# Autodesk Inventor assembly: Cadenas de soporte de bandejas 1.1
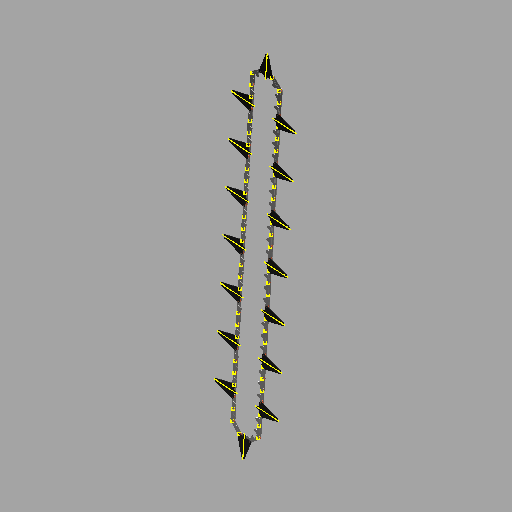
[picture p0: Inventor's stored thumbnail of the model, 512x512]
Saved by Autodesk Inventor 2024.3 (Build 283343010, 343A)
## iProperties
Created: 2025-05-22
Part Number: Cadenas de soporte de bandejas 1.1
Document SubType Name: Weldment
Designer: Gary
Weld Material: Welded Aluminum-6061
Author: Gary
## Documents named in this file (7)
- D:\OneDrive - Universidad Tecnologica del Peru\Desktop\Proyecto Final (Avance) Elementos de maquinas\Estructura principal\Cadenas de soporte de bandejas 1.1.iam
- D:\OneDrive - Universidad Tecnologica del Peru\Desktop\Proyecto Final (Avance) Elementos de maquinas\Estructura principal\Eslabon de arrastre posterior.ipt
- D:\OneDrive - Universidad Tecnologica del Peru\Desktop\Proyecto Final (Avance) Elementos de maquinas\Estructura principal\Eslabon de arrastre externo.ipt
- D:\OneDrive - Universidad Tecnologica del Peru\Desktop\Proyecto Final (Avance) Elementos de maquinas\Estructura principal\Eslabon de arrastre interno.ipt
- D:\OneDrive - Universidad Tecnologica del Peru\Desktop\Proyecto Final (Avance) Elementos de maquinas\Estructura principal\Rodillo Guia de Cadena.ipt
- D:\OneDrive - Universidad Tecnologica del Peru\Desktop\Proyecto Final (Avance) Elementos de maquinas\Estructura principal\Pasador Eslabones de Cadena.ipt
- D:\OneDrive - Universidad Tecnologica del Peru\Desktop\Proyecto Final (Avance) Elementos de maquinas\Estructura principal\Eslabon de arranque y movimiento bandeja.ipt
## Components (256 placed, 6 different names)
1. Eslabon de arrastre posterior:1 — Insert:12, Insert:13, Insert:16, Insert:283
2. Eslabon de arrastre externo:1 — Insert:4, Mate:1, Insert:6, Insert:7
3. Eslabon de arrastre interno:1 — Insert:3, Insert:4, Insert:5, Insert:353
4. Rodillo Guia de Cadena:1 — Insert:3, Insert:12
5. Pasador Eslabones de Cadena:1 — Insert:354
6. Pasador Eslabones de Cadena:2 — Insert:7
7. Pasador Eslabones de Cadena:3 — Mate:1
8. Pasador Eslabones de Cadena:4 — Insert:356
9. Rodillo Guia de Cadena:2 — Insert:5, Insert:13
10. Rodillo Guia de Cadena:3 — Insert:8, Insert:14
11. Rodillo Guia de Cadena:4 — Insert:11, Insert:15
12. Eslabon de arrastre interno:2 — Insert:6, Insert:8, Insert:11, Insert:355
13. Eslabon de arrastre posterior:2 — Insert:14, Insert:15, Insert:17, Insert:282
14. Eslabon de arrastre posterior:5 — Insert:16, Insert:17
15. Eslabon de arrastre posterior:9 — Insert:281
16. Eslabon de arrastre externo:2
17. Eslabon de arrastre interno:5 — Insert:357
18. Rodillo Guia de Cadena:9
19. Pasador Eslabones de Cadena:5 — Insert:358
20. Pasador Eslabones de Cadena:6
21. Pasador Eslabones de Cadena:7
22. Pasador Eslabones de Cadena:8 — Insert:360
23. Rodillo Guia de Cadena:10
24. Rodillo Guia de Cadena:11
25. Rodillo Guia de Cadena:12
26. Eslabon de arrastre interno:6 — Insert:359
27. Eslabon de arrastre posterior:10 — Insert:280
28. Eslabon de arrastre posterior:11
29. Eslabon de arrastre posterior:12 — Insert:279
30. Eslabon de arrastre externo:3
31. Eslabon de arrastre interno:7 — Insert:361
32. Rodillo Guia de Cadena:13
33. Pasador Eslabones de Cadena:9 — Insert:362
34. Pasador Eslabones de Cadena:10
35. Pasador Eslabones de Cadena:11
36. Pasador Eslabones de Cadena:12 — Insert:364
37. Rodillo Guia de Cadena:14
38. Rodillo Guia de Cadena:15
39. Rodillo Guia de Cadena:16
40. Eslabon de arrastre interno:8 — Insert:363
41. Eslabon de arrastre posterior:13 — Insert:278
42. Eslabon de arrastre posterior:14
43. Eslabon de arrastre posterior:15 — Insert:277
44. Eslabon de arrastre externo:4
45. Eslabon de arrastre interno:9 — Insert:365
46. Rodillo Guia de Cadena:17
47. Pasador Eslabones de Cadena:13
48. Pasador Eslabones de Cadena:14
49. Pasador Eslabones de Cadena:15 — Insert:303
50. Rodillo Guia de Cadena:18
51. Rodillo Guia de Cadena:19
52. Rodillo Guia de Cadena:20
53. Eslabon de arrastre interno:10 — Insert:306
54. Eslabon de arrastre posterior:16 — Insert:275
55. Eslabon de arrastre posterior:17
56. Eslabon de arrastre posterior:18 — Insert:276
57. Eslabon de arrastre externo:5
58. Eslabon de arrastre interno:11 — Insert:305
59. Rodillo Guia de Cadena:21
60. Pasador Eslabones de Cadena:16
61. Pasador Eslabones de Cadena:17
62. Pasador Eslabones de Cadena:18 — Insert:308
63. Rodillo Guia de Cadena:22
64. Rodillo Guia de Cadena:23
65. Rodillo Guia de Cadena:24
66. Eslabon de arrastre interno:12 — Insert:310
67. Eslabon de arrastre posterior:19 — Insert:273
68. Eslabon de arrastre posterior:20
69. Pasador Eslabones de Cadena:19 — Insert:366
70. Pasador Eslabones de Cadena:20 — Insert:304
71. Pasador Eslabones de Cadena:21 — Insert:352
72. Eslabon de arrastre posterior:21 — Insert:290
73. Eslabon de arrastre externo:6
74. Eslabon de arrastre interno:13 — Insert:332
75. Rodillo Guia de Cadena:25
76. Pasador Eslabones de Cadena:22 — Insert:334
77. Pasador Eslabones de Cadena:23
78. Pasador Eslabones de Cadena:24
79. Pasador Eslabones de Cadena:25 — Insert:336
80. Rodillo Guia de Cadena:26
81. Rodillo Guia de Cadena:27
82. Rodillo Guia de Cadena:28
83. Eslabon de arrastre interno:14 — Insert:335
84. Eslabon de arrastre posterior:22 — Mate:18
85. Eslabon de arrastre posterior:23
86. Eslabon de arrastre posterior:24 — Mate:17
87. Eslabon de arrastre externo:7
88. Eslabon de arrastre interno:15 — Insert:337
89. Rodillo Guia de Cadena:29
90. Pasador Eslabones de Cadena:26 — Insert:338
91. Pasador Eslabones de Cadena:27
92. Pasador Eslabones de Cadena:28
93. Pasador Eslabones de Cadena:29 — Insert:340
94. Rodillo Guia de Cadena:30
95. Rodillo Guia de Cadena:31
96. Rodillo Guia de Cadena:32
97. Eslabon de arrastre interno:16 — Insert:339
98. Eslabon de arrastre posterior:25 — Insert:288
99. Eslabon de arrastre posterior:26
100. Eslabon de arrastre posterior:27 — Insert:289
101. Eslabon de arrastre externo:8
102. Eslabon de arrastre interno:17 — Insert:341
103. Rodillo Guia de Cadena:33
104. Pasador Eslabones de Cadena:30 — Insert:342
105. Pasador Eslabones de Cadena:31
106. Pasador Eslabones de Cadena:32
107. Pasador Eslabones de Cadena:33 — Insert:344
108. Rodillo Guia de Cadena:34
109. Rodillo Guia de Cadena:35
110. Rodillo Guia de Cadena:36
111. Eslabon de arrastre interno:18 — Insert:343
112. Eslabon de arrastre posterior:28 — Insert:286
113. Eslabon de arrastre posterior:29
114. Eslabon de arrastre posterior:30 — Insert:287
115. Eslabon de arrastre externo:9
116. Eslabon de arrastre interno:19 — Insert:345
117. Rodillo Guia de Cadena:37
118. Pasador Eslabones de Cadena:34
119. Pasador Eslabones de Cadena:35
120. Pasador Eslabones de Cadena:36 — Insert:348
121. Rodillo Guia de Cadena:38
122. Rodillo Guia de Cadena:39
123. Rodillo Guia de Cadena:40
124. Eslabon de arrastre interno:20 — Insert:347
125. Eslabon de arrastre posterior:31 — Insert:284
126. Eslabon de arrastre posterior:32
127. Eslabon de arrastre posterior:33 — Insert:285
128. Eslabon de arrastre externo:10
129. Eslabon de arrastre interno:21 — Insert:349
130. Rodillo Guia de Cadena:41
131. Pasador Eslabones de Cadena:37
132. Pasador Eslabones de Cadena:38
133. Rodillo Guia de Cadena:42
134. Rodillo Guia de Cadena:43
135. Rodillo Guia de Cadena:44
136. Eslabon de arrastre interno:22 — Insert:351
137. Eslabon de arrastre posterior:34 — Insert:300
138. Eslabon de arrastre posterior:35
139. Pasador Eslabones de Cadena:39 — Insert:346
140. Pasador Eslabones de Cadena:40 — Insert:350
141. Eslabon de arrastre posterior:36 — Insert:302
142. Eslabon de arrastre externo:11
143. Eslabon de arrastre interno:23 — Insert:313
144. Rodillo Guia de Cadena:45
145. Pasador Eslabones de Cadena:41 — Insert:312
146. Pasador Eslabones de Cadena:42
147. Pasador Eslabones de Cadena:43
148. Pasador Eslabones de Cadena:44 — Insert:317
149. Rodillo Guia de Cadena:46
150. Rodillo Guia de Cadena:47
151. Rodillo Guia de Cadena:48
152. Eslabon de arrastre interno:24 — Insert:315
153. Eslabon de arrastre posterior:37 — Insert:299
154. Eslabon de arrastre posterior:38
155. Eslabon de arrastre posterior:39 — Insert:298
156. Eslabon de arrastre externo:12
157. Eslabon de arrastre interno:25 — Insert:316
158. Rodillo Guia de Cadena:49
159. Pasador Eslabones de Cadena:45 — Insert:318
160. Pasador Eslabones de Cadena:46
161. Pasador Eslabones de Cadena:47
162. Pasador Eslabones de Cadena:48 — Insert:321
163. Rodillo Guia de Cadena:50
164. Rodillo Guia de Cadena:51
165. Rodillo Guia de Cadena:52
166. Eslabon de arrastre interno:26 — Insert:319
167. Eslabon de arrastre posterior:40 — Insert:297
168. Eslabon de arrastre posterior:41
169. Eslabon de arrastre posterior:42 — Insert:296
170. Eslabon de arrastre externo:13
171. Eslabon de arrastre interno:27 — Insert:320
172. Rodillo Guia de Cadena:53
173. Pasador Eslabones de Cadena:49 — Insert:322
174. Pasador Eslabones de Cadena:50
175. Pasador Eslabones de Cadena:51
176. Pasador Eslabones de Cadena:52 — Insert:324
177. Rodillo Guia de Cadena:54
178. Rodillo Guia de Cadena:55
179. Rodillo Guia de Cadena:56
180. Eslabon de arrastre interno:28 — Insert:323
181. Eslabon de arrastre posterior:43 — Insert:295
182. Eslabon de arrastre posterior:44
183. Eslabon de arrastre posterior:45 — Insert:294
184. Eslabon de arrastre externo:14
185. Eslabon de arrastre interno:29 — Insert:325
186. Rodillo Guia de Cadena:57
187. Pasador Eslabones de Cadena:53
188. Pasador Eslabones de Cadena:54
189. Pasador Eslabones de Cadena:55 — Insert:329
190. Rodillo Guia de Cadena:58
191. Rodillo Guia de Cadena:59
192. Rodillo Guia de Cadena:60
193. Eslabon de arrastre interno:30 — Insert:327
194. Eslabon de arrastre posterior:46 — Insert:293
195. Eslabon de arrastre posterior:47
196. Eslabon de arrastre posterior:48 — Insert:292
197. Eslabon de arrastre externo:15
198. Eslabon de arrastre interno:31 — Insert:328
199. Rodillo Guia de Cadena:61
200. Pasador Eslabones de Cadena:56
201. Pasador Eslabones de Cadena:57
202. Rodillo Guia de Cadena:62
203. Rodillo Guia de Cadena:63
204. Rodillo Guia de Cadena:64
205. Eslabon de arrastre interno:32 — Insert:331
206. Eslabon de arrastre posterior:49 — Insert:291
207. Eslabon de arrastre posterior:50
208. Pasador Eslabones de Cadena:58 — Insert:326
209. Pasador Eslabones de Cadena:59 — Insert:330
210. Eslabon de arrastre posterior:51 — Insert:274
211. Eslabon de arrastre externo:16
212. Eslabon de arrastre interno:33 — Insert:309
213. Rodillo Guia de Cadena:66
214. Pasador Eslabones de Cadena:61
215. Pasador Eslabones de Cadena:62
216. Rodillo Guia de Cadena:67
217. Rodillo Guia de Cadena:68
218. Rodillo Guia de Cadena:69
219. Eslabon de arrastre interno:34 — Insert:314
220. Eslabon de arrastre posterior:52 — Insert:301
221. Eslabon de arrastre posterior:53
222. Pasador Eslabones de Cadena:63 — Insert:307
223. Eslabon de arrastre posterior:54 — Insert:273, Insert:274
224. Eslabon de arrastre posterior:55 — Insert:275, Insert:276
225. Eslabon de arrastre posterior:56 — Insert:277, Insert:278
226. Eslabon de arrastre posterior:57 — Insert:279, Insert:280
227. Eslabon de arrastre posterior:58 — Insert:281, Insert:282
228. Eslabon de arrastre posterior:59 — Insert:283, Insert:300
229. Eslabon de arrastre posterior:60 — Insert:284, Insert:285
230. Eslabon de arrastre posterior:61 — Insert:286, Insert:287
231. Eslabon de arrastre posterior:62 — Insert:288, Insert:289
232. Eslabon de arrastre posterior:63 — Mate:17, Mate:18
233. Eslabon de arrastre posterior:64 — Insert:290, Insert:291
234. Eslabon de arrastre posterior:65 — Insert:292, Insert:293
235. Eslabon de arrastre posterior:66 — Insert:294, Insert:295
236. Eslabon de arrastre posterior:67 — Insert:296, Insert:297
237. Eslabon de arrastre posterior:68 — Insert:298, Insert:299
238. Pasador Eslabones de Cadena:64 — Insert:333
239. Pasador Eslabones de Cadena:65 — Insert:311
240. Eslabon de arrastre posterior:69 — Insert:301, Insert:302
241. Eslabon de arranque y movimiento bandeja:1 — Insert:303, Insert:304, Insert:305, Insert:306
242. Eslabon de arranque y movimiento bandeja:2 — Insert:307, Insert:308, Insert:309, Insert:310
243. Eslabon de arranque y movimiento bandeja:3 — Insert:311, Insert:312, Insert:313, Insert:314
244. Eslabon de arranque y movimiento bandeja:4 — Insert:315, Insert:316, Insert:317, Insert:318
245. Eslabon de arranque y movimiento bandeja:5 — Insert:319, Insert:320, Insert:321, Insert:322
246. Eslabon de arranque y movimiento bandeja:6 — Insert:323, Insert:324, Insert:325, Insert:326
247. Eslabon de arranque y movimiento bandeja:7 — Insert:327, Insert:328, Insert:329, Insert:330
248. Eslabon de arranque y movimiento bandeja:8 — Insert:331, Insert:332, Insert:333, Insert:334
249. Eslabon de arranque y movimiento bandeja:9 — Insert:335, Insert:336, Insert:337, Insert:338
250. Eslabon de arranque y movimiento bandeja:10 — Insert:339, Insert:340, Insert:341, Insert:342
251. Eslabon de arranque y movimiento bandeja:11 — Insert:343, Insert:344, Insert:345, Insert:346
252. Eslabon de arranque y movimiento bandeja:12 — Insert:347, Insert:348, Insert:349, Insert:350
253. Eslabon de arranque y movimiento bandeja:13 — Insert:351, Insert:352, Insert:353, Insert:354
254. Eslabon de arranque y movimiento bandeja:14 — Insert:355, Insert:356, Insert:357, Insert:358
255. Eslabon de arranque y movimiento bandeja:15 — Insert:359, Insert:360, Insert:361, Insert:362
256. Eslabon de arranque y movimiento bandeja:16 — Insert:363, Insert:364, Insert:365, Insert:366
## Relationships (320: Insert 302, Mate 18)
- Insert:3: Eslabon de arrastre interno:1 ↔ Rodillo Guia de Cadena:1
- Insert:4: Eslabon de arrastre externo:1 ↔ Eslabon de arrastre interno:1
- Mate:1: Eslabon de arrastre externo:1 ↔ Pasador Eslabones de Cadena:3
- Insert:5: Eslabon de arrastre interno:1 ↔ Rodillo Guia de Cadena:2
- Insert:6: Eslabon de arrastre externo:1 ↔ Eslabon de arrastre interno:2
- Insert:7: Eslabon de arrastre externo:1 ↔ Pasador Eslabones de Cadena:2
- Insert:8: Rodillo Guia de Cadena:3 ↔ Eslabon de arrastre interno:2
- Insert:11: Rodillo Guia de Cadena:4 ↔ Eslabon de arrastre interno:2
- Insert:12: Eslabon de arrastre posterior:1 ↔ Rodillo Guia de Cadena:1
- Insert:13: Eslabon de arrastre posterior:1 ↔ Rodillo Guia de Cadena:2
- Insert:14: Rodillo Guia de Cadena:3 ↔ Eslabon de arrastre posterior:2
- Insert:15: Rodillo Guia de Cadena:4 ↔ Eslabon de arrastre posterior:2
- Insert:16: Eslabon de arrastre posterior:1 ↔ Eslabon de arrastre posterior:5
- Insert:17: Eslabon de arrastre posterior:2 ↔ Eslabon de arrastre posterior:5
- [Insert]: Eslabon de arrastre interno:5 ↔ Rodillo Guia de Cadena:9
- [Insert]: Eslabon de arrastre externo:2 ↔ Eslabon de arrastre interno:5
- [Mate]: Eslabon de arrastre externo:2 ↔ Pasador Eslabones de Cadena:7
- [Insert]: Eslabon de arrastre interno:5 ↔ Rodillo Guia de Cadena:10
- [Insert]: Eslabon de arrastre externo:2 ↔ Eslabon de arrastre interno:6
- [Insert]: Eslabon de arrastre externo:2 ↔ Pasador Eslabones de Cadena:6
- [Insert]: Rodillo Guia de Cadena:11 ↔ Eslabon de arrastre interno:6
- [Insert]: Rodillo Guia de Cadena:12 ↔ Eslabon de arrastre interno:6
- [Insert]: Eslabon de arrastre posterior:9 ↔ Rodillo Guia de Cadena:9
- [Insert]: Eslabon de arrastre posterior:9 ↔ Rodillo Guia de Cadena:10
- [Insert]: Rodillo Guia de Cadena:11 ↔ Eslabon de arrastre posterior:10
- [Insert]: Rodillo Guia de Cadena:12 ↔ Eslabon de arrastre posterior:10
- [Insert]: Eslabon de arrastre posterior:9 ↔ Eslabon de arrastre posterior:11
- [Insert]: Eslabon de arrastre posterior:10 ↔ Eslabon de arrastre posterior:11
- [Insert]: Eslabon de arrastre interno:7 ↔ Rodillo Guia de Cadena:13
- [Insert]: Eslabon de arrastre externo:3 ↔ Eslabon de arrastre interno:7
- [Mate]: Eslabon de arrastre externo:3 ↔ Pasador Eslabones de Cadena:11
- [Insert]: Eslabon de arrastre interno:7 ↔ Rodillo Guia de Cadena:14
- [Insert]: Eslabon de arrastre externo:3 ↔ Eslabon de arrastre interno:8
- [Insert]: Eslabon de arrastre externo:3 ↔ Pasador Eslabones de Cadena:10
- [Insert]: Rodillo Guia de Cadena:15 ↔ Eslabon de arrastre interno:8
- [Insert]: Rodillo Guia de Cadena:16 ↔ Eslabon de arrastre interno:8
- [Insert]: Eslabon de arrastre posterior:12 ↔ Rodillo Guia de Cadena:13
- [Insert]: Eslabon de arrastre posterior:12 ↔ Rodillo Guia de Cadena:14
- [Insert]: Rodillo Guia de Cadena:15 ↔ Eslabon de arrastre posterior:13
- [Insert]: Rodillo Guia de Cadena:16 ↔ Eslabon de arrastre posterior:13
- [Insert]: Eslabon de arrastre posterior:12 ↔ Eslabon de arrastre posterior:14
- [Insert]: Eslabon de arrastre posterior:13 ↔ Eslabon de arrastre posterior:14
- [Insert]: Eslabon de arrastre interno:9 ↔ Rodillo Guia de Cadena:17
- [Insert]: Eslabon de arrastre externo:4 ↔ Eslabon de arrastre interno:9
- [Mate]: Eslabon de arrastre externo:4 ↔ Pasador Eslabones de Cadena:14
- [Insert]: Eslabon de arrastre interno:9 ↔ Rodillo Guia de Cadena:18
- [Insert]: Eslabon de arrastre externo:4 ↔ Eslabon de arrastre interno:10
- [Insert]: Eslabon de arrastre externo:4 ↔ Pasador Eslabones de Cadena:13
- [Insert]: Rodillo Guia de Cadena:19 ↔ Eslabon de arrastre interno:10
- [Insert]: Rodillo Guia de Cadena:20 ↔ Eslabon de arrastre interno:10
- [Insert]: Eslabon de arrastre posterior:15 ↔ Rodillo Guia de Cadena:17
- [Insert]: Eslabon de arrastre posterior:15 ↔ Rodillo Guia de Cadena:18
- [Insert]: Rodillo Guia de Cadena:19 ↔ Eslabon de arrastre posterior:16
- [Insert]: Rodillo Guia de Cadena:20 ↔ Eslabon de arrastre posterior:16
- [Insert]: Eslabon de arrastre posterior:15 ↔ Eslabon de arrastre posterior:17
- [Insert]: Eslabon de arrastre posterior:16 ↔ Eslabon de arrastre posterior:17
- [Insert]: Eslabon de arrastre interno:11 ↔ Rodillo Guia de Cadena:21
- [Insert]: Eslabon de arrastre externo:5 ↔ Eslabon de arrastre interno:11
- [Mate]: Eslabon de arrastre externo:5 ↔ Pasador Eslabones de Cadena:17
- [Insert]: Eslabon de arrastre interno:11 ↔ Rodillo Guia de Cadena:22
- [Insert]: Eslabon de arrastre externo:5 ↔ Eslabon de arrastre interno:12
- [Insert]: Eslabon de arrastre externo:5 ↔ Pasador Eslabones de Cadena:16
- [Insert]: Rodillo Guia de Cadena:23 ↔ Eslabon de arrastre interno:12
- [Insert]: Rodillo Guia de Cadena:24 ↔ Eslabon de arrastre interno:12
- [Insert]: Eslabon de arrastre posterior:18 ↔ Rodillo Guia de Cadena:21
- [Insert]: Eslabon de arrastre posterior:18 ↔ Rodillo Guia de Cadena:22
- [Insert]: Rodillo Guia de Cadena:23 ↔ Eslabon de arrastre posterior:19
- [Insert]: Rodillo Guia de Cadena:24 ↔ Eslabon de arrastre posterior:19
- [Insert]: Eslabon de arrastre posterior:18 ↔ Eslabon de arrastre posterior:20
- [Insert]: Eslabon de arrastre posterior:19 ↔ Eslabon de arrastre posterior:20
- [Insert]: Eslabon de arrastre interno:13 ↔ Rodillo Guia de Cadena:25
- [Insert]: Eslabon de arrastre externo:6 ↔ Eslabon de arrastre interno:13
- [Mate]: Eslabon de arrastre externo:6 ↔ Pasador Eslabones de Cadena:24
- [Insert]: Eslabon de arrastre interno:13 ↔ Rodillo Guia de Cadena:26
- [Insert]: Eslabon de arrastre externo:6 ↔ Eslabon de arrastre interno:14
- [Insert]: Eslabon de arrastre externo:6 ↔ Pasador Eslabones de Cadena:23
- [Insert]: Rodillo Guia de Cadena:27 ↔ Eslabon de arrastre interno:14
- [Insert]: Rodillo Guia de Cadena:28 ↔ Eslabon de arrastre interno:14
- [Insert]: Eslabon de arrastre posterior:21 ↔ Rodillo Guia de Cadena:25
- [Insert]: Eslabon de arrastre posterior:21 ↔ Rodillo Guia de Cadena:26
- [Insert]: Rodillo Guia de Cadena:27 ↔ Eslabon de arrastre posterior:22
- [Insert]: Rodillo Guia de Cadena:28 ↔ Eslabon de arrastre posterior:22
- [Insert]: Eslabon de arrastre posterior:21 ↔ Eslabon de arrastre posterior:23
- [Insert]: Eslabon de arrastre posterior:22 ↔ Eslabon de arrastre posterior:23
- [Insert]: Eslabon de arrastre interno:15 ↔ Rodillo Guia de Cadena:29
- [Insert]: Eslabon de arrastre externo:7 ↔ Eslabon de arrastre interno:15
- [Mate]: Eslabon de arrastre externo:7 ↔ Pasador Eslabones de Cadena:28
- [Insert]: Eslabon de arrastre interno:15 ↔ Rodillo Guia de Cadena:30
- [Insert]: Eslabon de arrastre externo:7 ↔ Eslabon de arrastre interno:16
- [Insert]: Eslabon de arrastre externo:7 ↔ Pasador Eslabones de Cadena:27
- [Insert]: Rodillo Guia de Cadena:31 ↔ Eslabon de arrastre interno:16
- [Insert]: Rodillo Guia de Cadena:32 ↔ Eslabon de arrastre interno:16
- [Insert]: Eslabon de arrastre posterior:24 ↔ Rodillo Guia de Cadena:29
- [Insert]: Eslabon de arrastre posterior:24 ↔ Rodillo Guia de Cadena:30
- [Insert]: Rodillo Guia de Cadena:31 ↔ Eslabon de arrastre posterior:25
- [Insert]: Rodillo Guia de Cadena:32 ↔ Eslabon de arrastre posterior:25
- [Insert]: Eslabon de arrastre posterior:24 ↔ Eslabon de arrastre posterior:26
- [Insert]: Eslabon de arrastre posterior:25 ↔ Eslabon de arrastre posterior:26
- [Insert]: Eslabon de arrastre interno:17 ↔ Rodillo Guia de Cadena:33
- [Insert]: Eslabon de arrastre externo:8 ↔ Eslabon de arrastre interno:17
- [Mate]: Eslabon de arrastre externo:8 ↔ Pasador Eslabones de Cadena:32
- [Insert]: Eslabon de arrastre interno:17 ↔ Rodillo Guia de Cadena:34
- [Insert]: Eslabon de arrastre externo:8 ↔ Eslabon de arrastre interno:18
- [Insert]: Eslabon de arrastre externo:8 ↔ Pasador Eslabones de Cadena:31
- [Insert]: Rodillo Guia de Cadena:35 ↔ Eslabon de arrastre interno:18
- [Insert]: Rodillo Guia de Cadena:36 ↔ Eslabon de arrastre interno:18
- [Insert]: Eslabon de arrastre posterior:27 ↔ Rodillo Guia de Cadena:33
- [Insert]: Eslabon de arrastre posterior:27 ↔ Rodillo Guia de Cadena:34
- [Insert]: Rodillo Guia de Cadena:35 ↔ Eslabon de arrastre posterior:28
- [Insert]: Rodillo Guia de Cadena:36 ↔ Eslabon de arrastre posterior:28
- [Insert]: Eslabon de arrastre posterior:27 ↔ Eslabon de arrastre posterior:29
- [Insert]: Eslabon de arrastre posterior:28 ↔ Eslabon de arrastre posterior:29
- [Insert]: Eslabon de arrastre interno:19 ↔ Rodillo Guia de Cadena:37
- [Insert]: Eslabon de arrastre externo:9 ↔ Eslabon de arrastre interno:19
- [Mate]: Eslabon de arrastre externo:9 ↔ Pasador Eslabones de Cadena:35
- [Insert]: Eslabon de arrastre interno:19 ↔ Rodillo Guia de Cadena:38
- [Insert]: Eslabon de arrastre externo:9 ↔ Eslabon de arrastre interno:20
- [Insert]: Eslabon de arrastre externo:9 ↔ Pasador Eslabones de Cadena:34
- [Insert]: Rodillo Guia de Cadena:39 ↔ Eslabon de arrastre interno:20
- [Insert]: Rodillo Guia de Cadena:40 ↔ Eslabon de arrastre interno:20
- [Insert]: Eslabon de arrastre posterior:30 ↔ Rodillo Guia de Cadena:37
- [Insert]: Eslabon de arrastre posterior:30 ↔ Rodillo Guia de Cadena:38
- [Insert]: Rodillo Guia de Cadena:39 ↔ Eslabon de arrastre posterior:31
- [Insert]: Rodillo Guia de Cadena:40 ↔ Eslabon de arrastre posterior:31
- [Insert]: Eslabon de arrastre posterior:30 ↔ Eslabon de arrastre posterior:32
- [Insert]: Eslabon de arrastre posterior:31 ↔ Eslabon de arrastre posterior:32
- [Insert]: Eslabon de arrastre interno:21 ↔ Rodillo Guia de Cadena:41
- [Insert]: Eslabon de arrastre externo:10 ↔ Eslabon de arrastre interno:21
- [Mate]: Eslabon de arrastre externo:10 ↔ Pasador Eslabones de Cadena:38
- [Insert]: Eslabon de arrastre interno:21 ↔ Rodillo Guia de Cadena:42
- [Insert]: Eslabon de arrastre externo:10 ↔ Eslabon de arrastre interno:22
- [Insert]: Eslabon de arrastre externo:10 ↔ Pasador Eslabones de Cadena:37
- [Insert]: Rodillo Guia de Cadena:43 ↔ Eslabon de arrastre interno:22
- [Insert]: Rodillo Guia de Cadena:44 ↔ Eslabon de arrastre interno:22
- [Insert]: Eslabon de arrastre posterior:33 ↔ Rodillo Guia de Cadena:41
- [Insert]: Eslabon de arrastre posterior:33 ↔ Rodillo Guia de Cadena:42
- [Insert]: Rodillo Guia de Cadena:43 ↔ Eslabon de arrastre posterior:34
- [Insert]: Rodillo Guia de Cadena:44 ↔ Eslabon de arrastre posterior:34
- [Insert]: Eslabon de arrastre posterior:33 ↔ Eslabon de arrastre posterior:35
- [Insert]: Eslabon de arrastre posterior:34 ↔ Eslabon de arrastre posterior:35
- [Insert]: Eslabon de arrastre interno:23 ↔ Rodillo Guia de Cadena:45
- [Insert]: Eslabon de arrastre externo:11 ↔ Eslabon de arrastre interno:23
- [Mate]: Eslabon de arrastre externo:11 ↔ Pasador Eslabones de Cadena:43
- [Insert]: Eslabon de arrastre interno:23 ↔ Rodillo Guia de Cadena:46
- [Insert]: Eslabon de arrastre externo:11 ↔ Eslabon de arrastre interno:24
- [Insert]: Eslabon de arrastre externo:11 ↔ Pasador Eslabones de Cadena:42
- [Insert]: Rodillo Guia de Cadena:47 ↔ Eslabon de arrastre interno:24
- [Insert]: Rodillo Guia de Cadena:48 ↔ Eslabon de arrastre interno:24
- [Insert]: Eslabon de arrastre posterior:36 ↔ Rodillo Guia de Cadena:45
- [Insert]: Eslabon de arrastre posterior:36 ↔ Rodillo Guia de Cadena:46
- [Insert]: Rodillo Guia de Cadena:47 ↔ Eslabon de arrastre posterior:37
- [Insert]: Rodillo Guia de Cadena:48 ↔ Eslabon de arrastre posterior:37
- [Insert]: Eslabon de arrastre posterior:36 ↔ Eslabon de arrastre posterior:38
- [Insert]: Eslabon de arrastre posterior:37 ↔ Eslabon de arrastre posterior:38
- [Insert]: Eslabon de arrastre interno:25 ↔ Rodillo Guia de Cadena:49
- [Insert]: Eslabon de arrastre externo:12 ↔ Eslabon de arrastre interno:25
- [Mate]: Eslabon de arrastre externo:12 ↔ Pasador Eslabones de Cadena:47
- [Insert]: Eslabon de arrastre interno:25 ↔ Rodillo Guia de Cadena:50
- [Insert]: Eslabon de arrastre externo:12 ↔ Eslabon de arrastre interno:26
- [Insert]: Eslabon de arrastre externo:12 ↔ Pasador Eslabones de Cadena:46
- [Insert]: Rodillo Guia de Cadena:51 ↔ Eslabon de arrastre interno:26
- [Insert]: Rodillo Guia de Cadena:52 ↔ Eslabon de arrastre interno:26
- [Insert]: Eslabon de arrastre posterior:39 ↔ Rodillo Guia de Cadena:49
- [Insert]: Eslabon de arrastre posterior:39 ↔ Rodillo Guia de Cadena:50
- [Insert]: Rodillo Guia de Cadena:51 ↔ Eslabon de arrastre posterior:40
- [Insert]: Rodillo Guia de Cadena:52 ↔ Eslabon de arrastre posterior:40
- [Insert]: Eslabon de arrastre posterior:39 ↔ Eslabon de arrastre posterior:41
- [Insert]: Eslabon de arrastre posterior:40 ↔ Eslabon de arrastre posterior:41
- [Insert]: Eslabon de arrastre interno:27 ↔ Rodillo Guia de Cadena:53
- [Insert]: Eslabon de arrastre externo:13 ↔ Eslabon de arrastre interno:27
- [Mate]: Eslabon de arrastre externo:13 ↔ Pasador Eslabones de Cadena:51
- [Insert]: Eslabon de arrastre interno:27 ↔ Rodillo Guia de Cadena:54
- [Insert]: Eslabon de arrastre externo:13 ↔ Eslabon de arrastre interno:28
- [Insert]: Eslabon de arrastre externo:13 ↔ Pasador Eslabones de Cadena:50
- [Insert]: Rodillo Guia de Cadena:55 ↔ Eslabon de arrastre interno:28
- [Insert]: Rodillo Guia de Cadena:56 ↔ Eslabon de arrastre interno:28
- [Insert]: Eslabon de arrastre posterior:42 ↔ Rodillo Guia de Cadena:53
- [Insert]: Eslabon de arrastre posterior:42 ↔ Rodillo Guia de Cadena:54
- [Insert]: Rodillo Guia de Cadena:55 ↔ Eslabon de arrastre posterior:43
- [Insert]: Rodillo Guia de Cadena:56 ↔ Eslabon de arrastre posterior:43
- [Insert]: Eslabon de arrastre posterior:42 ↔ Eslabon de arrastre posterior:44
- [Insert]: Eslabon de arrastre posterior:43 ↔ Eslabon de arrastre posterior:44
- [Insert]: Eslabon de arrastre interno:29 ↔ Rodillo Guia de Cadena:57
- [Insert]: Eslabon de arrastre externo:14 ↔ Eslabon de arrastre interno:29
- [Mate]: Eslabon de arrastre externo:14 ↔ Pasador Eslabones de Cadena:54
- [Insert]: Eslabon de arrastre interno:29 ↔ Rodillo Guia de Cadena:58
- [Insert]: Eslabon de arrastre externo:14 ↔ Eslabon de arrastre interno:30
- [Insert]: Eslabon de arrastre externo:14 ↔ Pasador Eslabones de Cadena:53
- [Insert]: Rodillo Guia de Cadena:59 ↔ Eslabon de arrastre interno:30
- [Insert]: Rodillo Guia de Cadena:60 ↔ Eslabon de arrastre interno:30
- [Insert]: Eslabon de arrastre posterior:45 ↔ Rodillo Guia de Cadena:57
- [Insert]: Eslabon de arrastre posterior:45 ↔ Rodillo Guia de Cadena:58
- [Insert]: Rodillo Guia de Cadena:59 ↔ Eslabon de arrastre posterior:46
- [Insert]: Rodillo Guia de Cadena:60 ↔ Eslabon de arrastre posterior:46
- [Insert]: Eslabon de arrastre posterior:45 ↔ Eslabon de arrastre posterior:47
- [Insert]: Eslabon de arrastre posterior:46 ↔ Eslabon de arrastre posterior:47
- [Insert]: Eslabon de arrastre interno:31 ↔ Rodillo Guia de Cadena:61
- [Insert]: Eslabon de arrastre externo:15 ↔ Eslabon de arrastre interno:31
- [Mate]: Eslabon de arrastre externo:15 ↔ Pasador Eslabones de Cadena:57
- [Insert]: Eslabon de arrastre interno:31 ↔ Rodillo Guia de Cadena:62
- [Insert]: Eslabon de arrastre externo:15 ↔ Eslabon de arrastre interno:32
- [Insert]: Eslabon de arrastre externo:15 ↔ Pasador Eslabones de Cadena:56
- [Insert]: Rodillo Guia de Cadena:63 ↔ Eslabon de arrastre interno:32
- [Insert]: Rodillo Guia de Cadena:64 ↔ Eslabon de arrastre interno:32
- [Insert]: Eslabon de arrastre posterior:48 ↔ Rodillo Guia de Cadena:61
- [Insert]: Eslabon de arrastre posterior:48 ↔ Rodillo Guia de Cadena:62
- [Insert]: Rodillo Guia de Cadena:63 ↔ Eslabon de arrastre posterior:49
- [Insert]: Rodillo Guia de Cadena:64 ↔ Eslabon de arrastre posterior:49
- [Insert]: Eslabon de arrastre posterior:48 ↔ Eslabon de arrastre posterior:50
- [Insert]: Eslabon de arrastre posterior:49 ↔ Eslabon de arrastre posterior:50
- [Insert]: Eslabon de arrastre interno:33 ↔ Rodillo Guia de Cadena:66
- [Insert]: Eslabon de arrastre externo:16 ↔ Eslabon de arrastre interno:33
- [Mate]: Eslabon de arrastre externo:16 ↔ Pasador Eslabones de Cadena:62
- [Insert]: Eslabon de arrastre interno:33 ↔ Rodillo Guia de Cadena:67
- [Insert]: Eslabon de arrastre externo:16 ↔ Eslabon de arrastre interno:34
- [Insert]: Eslabon de arrastre externo:16 ↔ Pasador Eslabones de Cadena:61
- [Insert]: Rodillo Guia de Cadena:68 ↔ Eslabon de arrastre interno:34
- [Insert]: Rodillo Guia de Cadena:69 ↔ Eslabon de arrastre interno:34
- [Insert]: Eslabon de arrastre posterior:51 ↔ Rodillo Guia de Cadena:66
- [Insert]: Eslabon de arrastre posterior:51 ↔ Rodillo Guia de Cadena:67
- [Insert]: Rodillo Guia de Cadena:68 ↔ Eslabon de arrastre posterior:52
- [Insert]: Rodillo Guia de Cadena:69 ↔ Eslabon de arrastre posterior:52
- [Insert]: Eslabon de arrastre posterior:51 ↔ Eslabon de arrastre posterior:53
- [Insert]: Eslabon de arrastre posterior:52 ↔ Eslabon de arrastre posterior:53
- Insert:273: Eslabon de arrastre posterior:19 ↔ Eslabon de arrastre posterior:54
- Insert:274: Eslabon de arrastre posterior:51 ↔ Eslabon de arrastre posterior:54
- Insert:275: Eslabon de arrastre posterior:16 ↔ Eslabon de arrastre posterior:55
- Insert:276: Eslabon de arrastre posterior:18 ↔ Eslabon de arrastre posterior:55
- Insert:277: Eslabon de arrastre posterior:15 ↔ Eslabon de arrastre posterior:56
- Insert:278: Eslabon de arrastre posterior:13 ↔ Eslabon de arrastre posterior:56
- Insert:279: Eslabon de arrastre posterior:12 ↔ Eslabon de arrastre posterior:57
- Insert:280: Eslabon de arrastre posterior:10 ↔ Eslabon de arrastre posterior:57
- Insert:281: Eslabon de arrastre posterior:9 ↔ Eslabon de arrastre posterior:58
- Insert:282: Eslabon de arrastre posterior:2 ↔ Eslabon de arrastre posterior:58
- Insert:283: Eslabon de arrastre posterior:1 ↔ Eslabon de arrastre posterior:59
- Insert:284: Eslabon de arrastre posterior:31 ↔ Eslabon de arrastre posterior:60
- Insert:285: Eslabon de arrastre posterior:33 ↔ Eslabon de arrastre posterior:60
- Insert:286: Eslabon de arrastre posterior:28 ↔ Eslabon de arrastre posterior:61
- Insert:287: Eslabon de arrastre posterior:30 ↔ Eslabon de arrastre posterior:61
- Insert:288: Eslabon de arrastre posterior:25 ↔ Eslabon de arrastre posterior:62
- Insert:289: Eslabon de arrastre posterior:27 ↔ Eslabon de arrastre posterior:62
- Mate:17: Eslabon de arrastre posterior:24 ↔ Eslabon de arrastre posterior:63
- Mate:18: Eslabon de arrastre posterior:22 ↔ Eslabon de arrastre posterior:63
- Insert:290: Eslabon de arrastre posterior:21 ↔ Eslabon de arrastre posterior:64
- Insert:291: Eslabon de arrastre posterior:49 ↔ Eslabon de arrastre posterior:64
- Insert:292: Eslabon de arrastre posterior:48 ↔ Eslabon de arrastre posterior:65
- Insert:293: Eslabon de arrastre posterior:46 ↔ Eslabon de arrastre posterior:65
- Insert:294: Eslabon de arrastre posterior:45 ↔ Eslabon de arrastre posterior:66
- Insert:295: Eslabon de arrastre posterior:43 ↔ Eslabon de arrastre posterior:66
- Insert:296: Eslabon de arrastre posterior:42 ↔ Eslabon de arrastre posterior:67
- Insert:297: Eslabon de arrastre posterior:40 ↔ Eslabon de arrastre posterior:67
- Insert:298: Eslabon de arrastre posterior:39 ↔ Eslabon de arrastre posterior:68
- Insert:299: Eslabon de arrastre posterior:37 ↔ Eslabon de arrastre posterior:68
- Insert:300: Eslabon de arrastre posterior:34 ↔ Eslabon de arrastre posterior:59
- Insert:301: Eslabon de arrastre posterior:52 ↔ Eslabon de arrastre posterior:69
- Insert:302: Eslabon de arrastre posterior:36 ↔ Eslabon de arrastre posterior:69
- Insert:303: Pasador Eslabones de Cadena:15 ↔ Eslabon de arranque y movimiento bandeja:1
- Insert:304: Pasador Eslabones de Cadena:20 ↔ Eslabon de arranque y movimiento bandeja:1
- Insert:305: Eslabon de arrastre interno:11 ↔ Eslabon de arranque y movimiento bandeja:1
- Insert:306: Eslabon de arrastre interno:10 ↔ Eslabon de arranque y movimiento bandeja:1
- Insert:307: Pasador Eslabones de Cadena:63 ↔ Eslabon de arranque y movimiento bandeja:2
- Insert:308: Pasador Eslabones de Cadena:18 ↔ Eslabon de arranque y movimiento bandeja:2
- Insert:309: Eslabon de arrastre interno:33 ↔ Eslabon de arranque y movimiento bandeja:2
- Insert:310: Eslabon de arrastre interno:12 ↔ Eslabon de arranque y movimiento bandeja:2
- Insert:311: Pasador Eslabones de Cadena:65 ↔ Eslabon de arranque y movimiento bandeja:3
- Insert:312: Pasador Eslabones de Cadena:41 ↔ Eslabon de arranque y movimiento bandeja:3
- Insert:313: Eslabon de arrastre interno:23 ↔ Eslabon de arranque y movimiento bandeja:3
- Insert:314: Eslabon de arrastre interno:34 ↔ Eslabon de arranque y movimiento bandeja:3
- Insert:315: Eslabon de arrastre interno:24 ↔ Eslabon de arranque y movimiento bandeja:4
- Insert:316: Eslabon de arrastre interno:25 ↔ Eslabon de arranque y movimiento bandeja:4
- Insert:317: Pasador Eslabones de Cadena:44 ↔ Eslabon de arranque y movimiento bandeja:4
- Insert:318: Pasador Eslabones de Cadena:45 ↔ Eslabon de arranque y movimiento bandeja:4
- Insert:319: Eslabon de arrastre interno:26 ↔ Eslabon de arranque y movimiento bandeja:5
- Insert:320: Eslabon de arrastre interno:27 ↔ Eslabon de arranque y movimiento bandeja:5
- Insert:321: Pasador Eslabones de Cadena:48 ↔ Eslabon de arranque y movimiento bandeja:5
- Insert:322: Pasador Eslabones de Cadena:49 ↔ Eslabon de arranque y movimiento bandeja:5
- Insert:323: Eslabon de arrastre interno:28 ↔ Eslabon de arranque y movimiento bandeja:6
- Insert:324: Pasador Eslabones de Cadena:52 ↔ Eslabon de arranque y movimiento bandeja:6
- Insert:325: Eslabon de arrastre interno:29 ↔ Eslabon de arranque y movimiento bandeja:6
- Insert:326: Pasador Eslabones de Cadena:58 ↔ Eslabon de arranque y movimiento bandeja:6
- Insert:327: Eslabon de arrastre interno:30 ↔ Eslabon de arranque y movimiento bandeja:7
- Insert:328: Eslabon de arrastre interno:31 ↔ Eslabon de arranque y movimiento bandeja:7
- Insert:329: Pasador Eslabones de Cadena:55 ↔ Eslabon de arranque y movimiento bandeja:7
- Insert:330: Pasador Eslabones de Cadena:59 ↔ Eslabon de arranque y movimiento bandeja:7
- Insert:331: Eslabon de arrastre interno:32 ↔ Eslabon de arranque y movimiento bandeja:8
- Insert:332: Eslabon de arrastre interno:13 ↔ Eslabon de arranque y movimiento bandeja:8
- Insert:333: Pasador Eslabones de Cadena:64 ↔ Eslabon de arranque y movimiento bandeja:8
- Insert:334: Pasador Eslabones de Cadena:22 ↔ Eslabon de arranque y movimiento bandeja:8
- Insert:335: Eslabon de arrastre interno:14 ↔ Eslabon de arranque y movimiento bandeja:9
- Insert:336: Pasador Eslabones de Cadena:25 ↔ Eslabon de arranque y movimiento bandeja:9
- Insert:337: Eslabon de arrastre interno:15 ↔ Eslabon de arranque y movimiento bandeja:9
- Insert:338: Pasador Eslabones de Cadena:26 ↔ Eslabon de arranque y movimiento bandeja:9
- Insert:339: Eslabon de arrastre interno:16 ↔ Eslabon de arranque y movimiento bandeja:10
- Insert:340: Pasador Eslabones de Cadena:29 ↔ Eslabon de arranque y movimiento bandeja:10
- Insert:341: Eslabon de arrastre interno:17 ↔ Eslabon de arranque y movimiento bandeja:10
- Insert:342: Pasador Eslabones de Cadena:30 ↔ Eslabon de arranque y movimiento bandeja:10
- Insert:343: Eslabon de arrastre interno:18 ↔ Eslabon de arranque y movimiento bandeja:11
- Insert:344: Pasador Eslabones de Cadena:33 ↔ Eslabon de arranque y movimiento bandeja:11
- Insert:345: Eslabon de arrastre interno:19 ↔ Eslabon de arranque y movimiento bandeja:11
- Insert:346: Pasador Eslabones de Cadena:39 ↔ Eslabon de arranque y movimiento bandeja:11
- Insert:347: Eslabon de arrastre interno:20 ↔ Eslabon de arranque y movimiento bandeja:12
- Insert:348: Pasador Eslabones de Cadena:36 ↔ Eslabon de arranque y movimiento bandeja:12
- Insert:349: Eslabon de arrastre interno:21 ↔ Eslabon de arranque y movimiento bandeja:12
- Insert:350: Pasador Eslabones de Cadena:40 ↔ Eslabon de arranque y movimiento bandeja:12
- Insert:351: Eslabon de arrastre interno:22 ↔ Eslabon de arranque y movimiento bandeja:13
- Insert:352: Pasador Eslabones de Cadena:21 ↔ Eslabon de arranque y movimiento bandeja:13
- Insert:353: Eslabon de arrastre interno:1 ↔ Eslabon de arranque y movimiento bandeja:13
- Insert:354: Pasador Eslabones de Cadena:1 ↔ Eslabon de arranque y movimiento bandeja:13
- Insert:355: Eslabon de arrastre interno:2 ↔ Eslabon de arranque y movimiento bandeja:14
- Insert:356: Pasador Eslabones de Cadena:4 ↔ Eslabon de arranque y movimiento bandeja:14
- Insert:357: Eslabon de arrastre interno:5 ↔ Eslabon de arranque y movimiento bandeja:14
- Insert:358: Pasador Eslabones de Cadena:5 ↔ Eslabon de arranque y movimiento bandeja:14
- Insert:359: Eslabon de arrastre interno:6 ↔ Eslabon de arranque y movimiento bandeja:15
- Insert:360: Pasador Eslabones de Cadena:8 ↔ Eslabon de arranque y movimiento bandeja:15
- Insert:361: Eslabon de arrastre interno:7 ↔ Eslabon de arranque y movimiento bandeja:15
- Insert:362: Pasador Eslabones de Cadena:9 ↔ Eslabon de arranque y movimiento bandeja:15
- Insert:363: Eslabon de arrastre interno:8 ↔ Eslabon de arranque y movimiento bandeja:16
- Insert:364: Pasador Eslabones de Cadena:12 ↔ Eslabon de arranque y movimiento bandeja:16
- Insert:365: Eslabon de arrastre interno:9 ↔ Eslabon de arranque y movimiento bandeja:16
- Insert:366: Pasador Eslabones de Cadena:19 ↔ Eslabon de arranque y movimiento bandeja:16
## Named parameters: d21_d12 = 0 mm, d22_d13 = 0 mm, d23_d14 = 0 mm, d24_d15 = 0 mm, d25_d16 = 0 mm, d26_d17 = 0 mm, d27_d18 = 0 mm, d28_d3 = 0 mm, d29_d4 = 0 mm, d30_d5 = 0 mm, d31_d6 = 0 mm, d32_d7 = 0 mm, d33_d8 = 0 mm, d34_d9 = 0 mm, d41_d21_d12 = 0 mm, d42_d22_d13 = 0 mm, d43_d23_d14 = 0 mm, d44_d24_d15 = 0 mm, d45_d25_d16 = 0 mm, d46_d26_d17 = 0 mm, d47_d27_d18 = 0 mm, d48_d28_d3 = 0 mm, d49_d29_d4 = 0 mm, d50_d30_d5 = 0 mm, d51_d31_d6 = 0 mm, d52_d32_d7 = 0 mm, d53_d33_d8 = 0 mm, d54_d34_d9 = 0 mm, d58_d41_d21_d12 = 0 mm, d59_d42_d22_d13 = 0 mm, d60_d43_d23_d14 = 0 mm, d61_d44_d24_d15 = 0 mm, d62_d45_d25_d16 = 0 mm, d63_d46_d26_d17 = 0 mm, d64_d47_d27_d18 = 0 mm, d65_d48_d28_d3 = 0 mm, d66_d49_d29_d4 = 0 mm, d67_d50_d30_d5 = 0 mm, d68_d51_d31_d6 = 0 mm, d69_d52_d32_d7 = 0 mm, d70_d53_d33_d8 = 0 mm, d71_d54_d34_d9 = 0 mm, d75_d41_d21_d12 = 0 mm, d76_d42_d22_d13 = 0 mm, d77_d43_d23_d14 = 0 mm, d78_d44_d24_d15 = 0 mm, d79_d45_d25_d16 = 0 mm, d80_d46_d26_d17 = 0 mm, d81_d47_d27_d18 = 0 mm, d82_d48_d28_d3 = 0 mm, d83_d49_d29_d4 = 0 mm, d84_d50_d30_d5 = 0 mm, d85_d51_d31_d6 = 0 mm, d86_d52_d32_d7 = 0 mm, d87_d53_d33_d8 = 0 mm, d88_d54_d34_d9 = 0 mm, d100_d58_d41_d21_d12 = 0 mm, d101_d59_d42_d22_d13 = 0 mm, d102_d60_d43_d23_d14 = 0 mm, d103_d61_d44_d24_d15 = 0 mm, d104_d62_d45_d25_d16 = 0 mm, d105_d63_d46_d26_d17 = 0 mm, d106_d64_d47_d27_d18 = 0 mm, d107_d65_d48_d28_d3 = 0 mm, d108_d66_d49_d29_d4 = 0 mm, d109_d67_d50_d30_d5 = 0 mm, d110_d68_d51_d31_d6 = 0 mm, d111_d69_d52_d32_d7 = 0 mm, d112_d70_d53_d33_d8 = 0 mm, d113_d71_d54_d34_d9 = 0 mm, d115_d75_d41_d21_d12 = 0 mm, d116_d76_d42_d22_d13 = 0 mm, d117_d77_d43_d23_d14 = 0 mm, d118_d78_d44_d24_d15 = 0 mm, d119_d79_d45_d25_d16 = 0 mm, d120_d80_d46_d26_d17 = 0 mm, d121_d81_d47_d27_d18 = 0 mm, d122_d82_d48_d28_d3 = 0 mm, d123_d83_d49_d29_d4 = 0 mm, d124_d84_d50_d30_d5 = 0 mm, d125_d85_d51_d31_d6 = 0 mm, d126_d86_d52_d32_d7 = 0 mm, d127_d87_d53_d33_d8 = 0 mm, d128_d88_d54_d34_d9 = 0 mm, d133_d41_d21_d12 = 0 mm, d134_d42_d22_d13 = 0 mm, d135_d43_d23_d14 = 0 mm, d136_d44_d24_d15 = 0 mm, d137_d45_d25_d16 = 0 mm, d138_d46_d26_d17 = 0 mm, d139_d47_d27_d18 = 0 mm, d140_d48_d28_d3 = 0 mm, d141_d49_d29_d4 = 0 mm, d142_d50_d30_d5 = 0 mm, d143_d51_d31_d6 = 0 mm, d144_d52_d32_d7 = 0 mm, d145_d53_d33_d8 = 0 mm, d146_d54_d34_d9 = 0 mm, d149_d12 = 0 mm, d150_d13 = 0 mm, d151_d14 = 0 mm, d152_d15 = 0 mm, d153_d16 = 0 mm, d154_d17 = 0 mm, d155_d18 = 0 mm, d158_d21_d12 = 0 mm, d159_d22_d13 = 0 mm, d160_d23_d14 = 0 mm, d161_d24_d15 = 0 mm, d162_d25_d16 = 0 mm, d163_d26_d17 = 0 mm, d164_d27_d18 = 0 mm, d165_d28_d3 = 0 mm, d166_d29_d4 = 0 mm, d167_d30_d5 = 0 mm, d168_d31_d6 = 0 mm, d169_d32_d7 = 0 mm, d170_d33_d8 = 0 mm, d171_d34_d9 = 0 mm, d174_d3 = 0 mm, d175_d4 = 0 mm, d176_d5 = 0 mm, d177_d6 = 0 mm, d178_d7 = 0 mm, d179_d8 = 0 mm, d180_d9 = 0 mm, d188_d58_d41_d21_d12 = 0 mm, d189_d59_d42_d22_d13 = 0 mm, d190_d60_d43_d23_d14 = 0 mm, d191_d61_d44_d24_d15 = 0 mm, d192_d62_d45_d25_d16 = 0 mm, d193_d63_d46_d26_d17 = 0 mm, d194_d64_d47_d27_d18 = 0 mm, d195_d65_d48_d28_d3 = 0 mm, d196_d66_d49_d29_d4 = 0 mm, d197_d67_d50_d30_d5 = 0 mm, d198_d68_d51_d31_d6 = 0 mm, d199_d69_d52_d32_d7 = 0 mm, d200_d70_d53_d33_d8 = 0 mm, d201_d71_d54_d34_d9 = 0 mm, d203_d75_d41_d21_d12 = 0 mm, d204_d76_d42_d22_d13 = 0 mm, d205_d77_d43_d23_d14 = 0 mm, d206_d78_d44_d24_d15 = 0 mm, d207_d79_d45_d25_d16 = 0 mm, d208_d80_d46_d26_d17 = 0 mm, d209_d81_d47_d27_d18 = 0 mm, d210_d82_d48_d28_d3 = 0 mm, d211_d83_d49_d29_d4 = 0 mm, d212_d84_d50_d30_d5 = 0 mm, d213_d85_d51_d31_d6 = 0 mm, d214_d86_d52_d32_d7 = 0 mm, d215_d87_d53_d33_d8 = 0 mm, d216_d88_d54_d34_d9 = 0 mm, d221_d41_d21_d12 = 0 mm, d222_d42_d22_d13 = 0 mm, d223_d43_d23_d14 = 0 mm, d224_d44_d24_d15 = 0 mm, d225_d45_d25_d16 = 0 mm, d226_d46_d26_d17 = 0 mm, d227_d47_d27_d18 = 0 mm, d228_d48_d28_d3 = 0 mm, d229_d49_d29_d4 = 0 mm, d230_d50_d30_d5 = 0 mm, d231_d51_d31_d6 = 0 mm, d232_d52_d32_d7 = 0 mm, d233_d53_d33_d8 = 0 mm, d234_d54_d34_d9 = 0 mm, d237_d12 = 0 mm, d238_d13 = 0 mm, d239_d14 = 0 mm, d240_d15 = 0 mm, d241_d16 = 0 mm, d242_d17 = 0 mm, d243_d18 = 0 mm, d246_d21_d12 = 0 mm, d247_d22_d13 = 0 mm, d248_d23_d14 = 0 mm, d249_d24_d15 = 0 mm, d250_d25_d16 = 0 mm, d251_d26_d17 = 0 mm, d252_d27_d18 = 0 mm, d253_d28_d3 = 0 mm, d254_d29_d4 = 0 mm, d255_d30_d5 = 0 mm, d256_d31_d6 = 0 mm, d257_d32_d7 = 0 mm, d258_d33_d8 = 0 mm, d259_d34_d9 = 0 mm, d262_d3 = 0 mm, d263_d4 = 0 mm, d264_d5 = 0 mm, d265_d6 = 0 mm, d266_d7 = 0 mm, d267_d8 = 0 mm, d268_d9 = 0 mm, d274_d75_d41_d21_d12 = 0 mm, d275_d76_d42_d22_d13 = 0 mm, d276_d77_d43_d23_d14 = 0 mm, d277_d78_d44_d24_d15 = 0 mm, d278_d79_d45_d25_d16 = 0 mm, d279_d80_d46_d26_d17 = 0 mm, d280_d81_d47_d27_d18 = 0 mm, d281_d82_d48_d28_d3 = 0 mm, d282_d83_d49_d29_d4 = 0 mm, d283_d84_d50_d30_d5 = 0 mm, d284_d85_d51_d31_d6 = 0 mm, d285_d86_d52_d32_d7 = 0 mm, d286_d87_d53_d33_d8 = 0 mm, d287_d88_d54_d34_d9 = 0 mm
